# Autodesk Inventor assembly: Upper gearbox main assembly
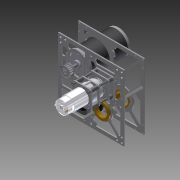
[picture p0: Inventor's stored thumbnail of the model, 180x180]
Saved by Autodesk Inventor 2012 (Build 160160000, 160)
## iProperties
Created: 2012-07-08
Part Number: Upper gearbox main assembly
Document SubType Name: Assembly
Designer: Bryce
Author: Bryce
## Documents named in this file (10)
- C:\Users\Bryce\Dropbox\Inventor Design Project Files\Independent Swerves\Inventor 2012\Upper gearbox main assembly.iam
- C:\Users\Bryce\Dropbox\Inventor Design Project Files\Independent Swerves\Inventor 2012\upper gearbox bottom plate.ipt
- C:\Users\Bryce\Dropbox\Inventor Design Project Files\Independent Swerves\Inventor 2012\upper gearbox top plate.ipt
- C:\Users\Bryce\Dropbox\Inventor Design Project Files\Independent Swerves\Imported Components\0.5'' 15 tooth flange threaded.ipt
- C:\Users\Bryce\Dropbox\Inventor Design Project Files\Independent Swerves\Imported Components\BD Gearbox and Bracket Assy 3.iam
- C:\Users\Bryce\Dropbox\Inventor Design Project Files\Independent Swerves\Inventor 2012\turn encoder assembly.iam
- C:\Users\Bryce\Dropbox\Inventor Design Project Files\Independent Swerves\Inventor 2012\collar bearing systom.ipt
- C:\Users\Bryce\Dropbox\Inventor Design Project Files\Independent Swerves\Inventor 2012\upper gearbox stand off standard.ipt
- C:\Users\Bryce\Dropbox\Inventor Design Project Files\Independent Swerves\Imported Components\CIM Motor.iam
- C:\Users\Bryce\Dropbox\Inventor Design Project Files\Independent Swerves\Imported Components\.375 15 tooth flange short.ipt
## Components (12 placed, 9 different names)
1. upper gearbox bottom plate:1 — Mate:74, Mate:75, Mate:108, Mate:109, Mate:110, Mate:111, Mate:112, Mate:113, Flush:4, Flush:5, Mate:129
2. upper gearbox top plate:1 — Mate:72, Mate:73, Mate:91, Mate:92, Mate:114, Mate:115, Mate:116, Mate:118, Mate:119, Mate:120, Mate:121, Mate:122, Mate:123, Mate:124, Angle:2, Mate:125, Mate:126, Mate:127, Mate:128, Flush:4, Flush:5, Mate:129
3. BD Gearbox and Bracket Assy 3:1 [sub-assembly] — Mate:56, Flush:3, Mate:125, Mate:126, Mate:127, Mate:128
4. 0.5'' 15 tooth flange threaded:2 — Mate:56, Flush:3
5. turn encoder assembly:1 [sub-assembly] — Mate:123, Mate:124, Angle:1, Angle:2
6. turn encoder assembly:2 [sub-assembly] — Mate:121, Mate:122, Angle:1
7. collar bearing systom:1 — Mate:74, Mate:75
8. collar bearing systom:2 — Mate:72, Mate:73, Mate:91, Mate:92
9. upper gearbox stand off standard:1 — Mate:108, Mate:109, Mate:110
10. upper gearbox stand off standard:2 — Mate:111, Mate:112, Mate:113
11. CIM Motor:1 [sub-assembly] — Mate:114, Mate:115, Mate:116, Mate:117, Mate:118, Mate:119, Mate:120
12. .375 15 tooth flange short:1 — Mate:117
## Relationships (34: Mate 29, Flush 3, Angle 2)
- Mate:56: BD Gearbox and Bracket Assy 3:1 ↔ 0.5'' 15 tooth flange threaded:2
- Flush:3: BD Gearbox and Bracket Assy 3:1 ↔ 0.5'' 15 tooth flange threaded:2
- Mate:72: upper gearbox top plate:1 ↔ collar bearing systom:2
- Mate:73: upper gearbox top plate:1 ↔ collar bearing systom:2
- Mate:74: upper gearbox bottom plate:1 ↔ collar bearing systom:1
- Mate:75: upper gearbox bottom plate:1 ↔ collar bearing systom:1
- Mate:91: upper gearbox top plate:1 ↔ collar bearing systom:2
- Mate:92: upper gearbox top plate:1 ↔ collar bearing systom:2
- Mate:108: upper gearbox bottom plate:1 ↔ upper gearbox stand off standard:1
- Mate:109: upper gearbox bottom plate:1 ↔ upper gearbox stand off standard:1
- Mate:110: upper gearbox bottom plate:1 ↔ upper gearbox stand off standard:1
- Mate:111: upper gearbox bottom plate:1 ↔ upper gearbox stand off standard:2
- Mate:112: upper gearbox bottom plate:1 ↔ upper gearbox stand off standard:2
- Mate:113: upper gearbox bottom plate:1 ↔ upper gearbox stand off standard:2
- Mate:114: upper gearbox top plate:1 ↔ CIM Motor:1
- Mate:115: upper gearbox top plate:1 ↔ CIM Motor:1
- Mate:116: upper gearbox top plate:1 ↔ CIM Motor:1
- Mate:117: CIM Motor:1 ↔ .375 15 tooth flange short:1
- Mate:118 (9.525 mm): upper gearbox top plate:1 ↔ CIM Motor:1
- Mate:119 (9.525 mm): upper gearbox top plate:1 ↔ CIM Motor:1
- Mate:120 (9.525 mm): upper gearbox top plate:1 ↔ CIM Motor:1
- Mate:121: upper gearbox top plate:1 ↔ turn encoder assembly:2
- Mate:122: upper gearbox top plate:1 ↔ turn encoder assembly:2
- Mate:123: upper gearbox top plate:1 ↔ turn encoder assembly:1
- Mate:124: upper gearbox top plate:1 ↔ turn encoder assembly:1
- Angle:1 (0 deg): turn encoder assembly:1 ↔ turn encoder assembly:2
- Angle:2 (0 deg): upper gearbox top plate:1 ↔ turn encoder assembly:1
- Mate:125: upper gearbox top plate:1 ↔ BD Gearbox and Bracket Assy 3:1
- Mate:126 (6.35 mm): upper gearbox top plate:1 ↔ BD Gearbox and Bracket Assy 3:1
- Mate:127 (6.35 mm): upper gearbox top plate:1 ↔ BD Gearbox and Bracket Assy 3:1
- Mate:128 (6.35 mm): upper gearbox top plate:1 ↔ BD Gearbox and Bracket Assy 3:1
- Flush:4: upper gearbox bottom plate:1 ↔ upper gearbox top plate:1
- Flush:5: upper gearbox bottom plate:1 ↔ upper gearbox top plate:1
- Mate:129 (50.8 mm): upper gearbox bottom plate:1 ↔ upper gearbox top plate:1
